# Autodesk Inventor assembly: ToiletBowl2.0Assembly
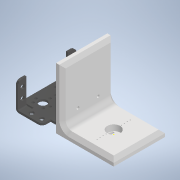
[picture p0: Inventor's stored thumbnail of the model, 180x180]
Saved by Autodesk Inventor 2020 (Build 240168000, 168)
## iProperties
Created: 2020-04-19
Part Number: ToiletBowl2.0Assembly
Document SubType Name: Assembly
Designer: Varun Kumar
Author: Varun Kumar
## Documents named in this file (3)
- C:\Users\Varun Kumar\Desktop\ServoArm\ToiletBowl2.0Assembly.iam
- C:\Users\Varun Kumar\Desktop\ServoArm\ToiletBowl2.0.ipt
- C:\Users\Varun Kumar\Desktop\ServoArm\Multi Purpose Bracket.ipt
## Components (2 placed, 2 different names)
1. ToiletBowl2.0:1 — Mate:1, Flush:1, Flush:2
2. Multi Purpose Bracket:1 — Mate:1, Flush:1, Flush:2
## Relationships (3: Flush 2, Mate 1)
- Mate:1: ToiletBowl2.0:1 ↔ Multi Purpose Bracket:1
- Flush:1 (4.9 mm): ToiletBowl2.0:1 ↔ Multi Purpose Bracket:1
- Flush:2 (31 mm): ToiletBowl2.0:1 ↔ Multi Purpose Bracket:1
